# Autodesk Inventor assembly: LCD
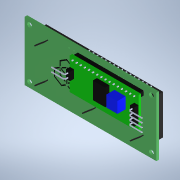
[picture p0: Inventor's stored thumbnail of the model, 180x180]
Saved by Autodesk Inventor 2022 (Build 260153000, 153)
## iProperties
Created: 2022-02-27
Part Number: LCD
Document SubType Name: Assembly
Designer: alexo
Author: alexo
## Documents named in this file (3)
- C:\Users\alexo\Documents\Inventor\Scanner3D\LCD.iam
- C:\Users\alexo\Documents\Inventor\Scanner3D\LCD_I2C_adapter.ipt
- C:\Users\alexo\Documents\Inventor\Scanner3D\LCD1602.ipt
## Components (2 placed, 2 different names)
1. LCD_I2C_adapter:1 — Rigid:1
2. LCD1602:1 — Rigid:1
## Relationships (1: WeldJoint 1)
- Rigid:1 [WeldJoint] (5 mm): LCD_I2C_adapter:1 ↔ LCD1602:1
